# Autodesk Inventor assembly: 160mmLens_assembly_table
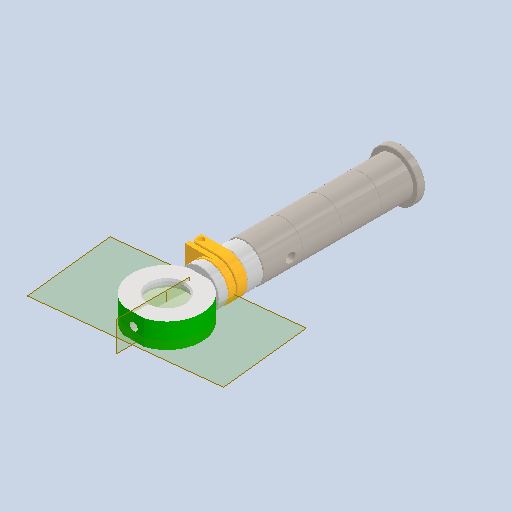
[picture p0: Inventor's stored thumbnail of the model, 512x512]
Saved by Autodesk Inventor 2026.1 (Build 301233000, 233)
## iProperties
Created: 2019-09-03
Part Number: 160mmLens_assembly_table
Document SubType Name: Assembly
Designer: Julian
Author: Julian
## Documents named in this file (7)
- C:\Users\user\Desktop\setup for publishing\160mmLens_assembly_table.iam
- C:\Users\user\Desktop\setup for publishing\M-PS-4_4in_ped_post.ipt
- C:\Users\user\Desktop\setup for publishing\25mmLensMount.ipt
- C:\Users\user\Desktop\setup for publishing\160 mm lens.iam
- C:\Users\user\Desktop\setup for publishing\M-PS-KF_miroor_flip.ipt
- C:\Users\user\Desktop\setup for publishing\RS10M-1in_10mm_post.ipt
- C:\Users\user\Desktop\setup for publishing\RS6M-6mm Spacer.ipt
## Components (6 placed, 6 different names)
1. M-PS-4_4in_ped_post:1 — Mate:1, Mate:2
2. 25mmLensMount:1 — Mate:7, Mate:8, Angle:1, Mate:9, Mate:10, Mate:11, Angle:2
3. 160 mm lens:1 [sub-assembly] — Mate:9, Mate:10
4. M-PS-KF_miroor_flip:1 — Mate:3, Mate:4, Mate:5, Mate:6, Angle:1
5. RS10M-1in_10mm_post:1 — Mate:1, Mate:2, Mate:3, Mate:4
6. RS6M-6mm Spacer:1 — Mate:5, Mate:6, Mate:7, Mate:8
## Relationships (14: Mate 12, Angle 2)
- Mate:1: M-PS-4_4in_ped_post:1 ↔ RS10M-1in_10mm_post:1
- Mate:2: M-PS-4_4in_ped_post:1 ↔ RS10M-1in_10mm_post:1
- Mate:3: M-PS-KF_miroor_flip:1 ↔ RS10M-1in_10mm_post:1
- Mate:4: M-PS-KF_miroor_flip:1 ↔ RS10M-1in_10mm_post:1
- Mate:5: M-PS-KF_miroor_flip:1 ↔ RS6M-6mm Spacer:1
- Mate:6: M-PS-KF_miroor_flip:1 ↔ RS6M-6mm Spacer:1
- Mate:7: 25mmLensMount:1 ↔ RS6M-6mm Spacer:1
- Mate:8: 25mmLensMount:1 ↔ RS6M-6mm Spacer:1
- Angle:1 (0 deg): 25mmLensMount:1 ↔ M-PS-KF_miroor_flip:1
- Mate:9: 25mmLensMount:1 ↔ 160 mm lens:1
- Mate:10 (-0.7 mm): 25mmLensMount:1 ↔ 160 mm lens:1
- Mate:11: 25mmLensMount:1
- Mate:12
- Angle:2 (90 deg): 25mmLensMount:1
